# Autodesk Inventor assembly: tail_p1
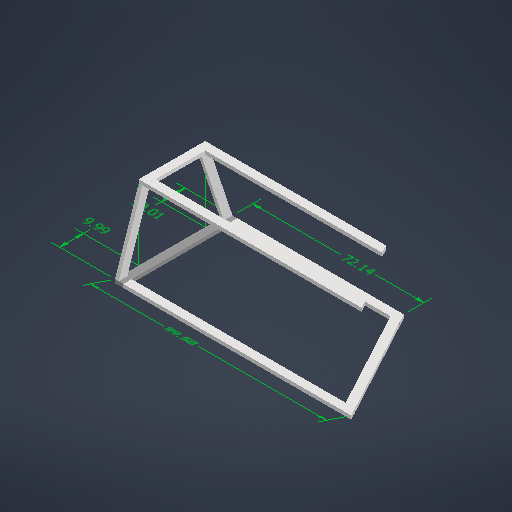
[picture p0: Inventor's stored thumbnail of the model, 512x512]
Saved by Autodesk Inventor 2027.1 (Build 311270010, 270A)
## iProperties
Created: 2026-09-01
Part Number: tail_p1
Document SubType Name: Assembly
Designer: jorda
Author: jorda
## Documents named in this file (9)
- C:\Users\jorda\OneDrive\Documents\GitHub\USC-ASME-TigerBurn-2026\CAD\Tail\tail_p1.iam
- C:\Users\jorda\OneDrive\Documents\GitHub\USC-ASME-TigerBurn-2026\CAD\Tail\2x4x48.ipt
- C:\Users\jorda\OneDrive\Documents\GitHub\USC-ASME-TigerBurn-2026\CAD\Tail\S_2x4x50.56.ipt
- C:\Users\jorda\OneDrive\Documents\GitHub\USC-ASME-TigerBurn-2026\CAD\Tail\S_2x4x72.ipt
- C:\Users\jorda\OneDrive\Documents\GitHub\USC-ASME-TigerBurn-2026\CAD\Tail\S_2x4x96.ipt
- C:\Users\jorda\OneDrive\Documents\GitHub\USC-ASME-TigerBurn-2026\CAD\Tail\S_2x4x32.93.ipt
- C:\Users\jorda\OneDrive\Documents\GitHub\USC-ASME-TigerBurn-2026\CAD\Tail\2x4x28.ipt
- C:\Users\jorda\OneDrive\Documents\GitHub\USC-ASME-TigerBurn-2026\CAD\Tail\S_2x4x93.85.ipt
- C:\Users\jorda\OneDrive\Documents\GitHub\USC-ASME-TigerBurn-2026\CAD\Tail\S_2x4x74.54.ipt
## Components (9 placed, 8 different names)
1. 2x4x48:1 — Mate:3, Flush:5, Flush:6, Mate:4, Flush:7, Flush:8, Mate:9, Flush:11, Mate:10, Flush:12
2. S_2x4x50.56:1
3. S_2x4x72:1 — Mate:3, Flush:5, Flush:6
4. S_2x4x96:1 — Mate:4, Flush:7, Flush:8
5. S_2x4x32.93:1 — Mate:9, Flush:11, Mate:11, Mate:12, Flush:13
6. S_2x4x32.93:2 — Mate:10, Flush:12
7. 2x4x28:1 — Mate:11, Mate:12, Flush:13, Mate:15, Flush:18, Flush:19, Mate:16, Flush:20, Flush:21, Mate:17, Flush:22, Flush:23
8. S_2x4x93.85:1 — Mate:15, Flush:18, Flush:19, Mate:16, Flush:20, Flush:21
9. S_2x4x74.54:1 — Mate:17, Flush:22, Flush:23
## Relationships (22: Flush 13, Mate 9)
- Mate:3: 2x4x48:1 ↔ S_2x4x72:1
- Flush:5: 2x4x48:1 ↔ S_2x4x72:1
- Flush:6: 2x4x48:1 ↔ S_2x4x72:1
- Mate:4: 2x4x48:1 ↔ S_2x4x96:1
- Flush:7: 2x4x48:1 ↔ S_2x4x96:1
- Flush:8: 2x4x48:1 ↔ S_2x4x96:1
- Mate:9: 2x4x48:1 ↔ S_2x4x32.93:1
- Flush:11: 2x4x48:1 ↔ S_2x4x32.93:1
- Mate:10: 2x4x48:1 ↔ S_2x4x32.93:2
- Flush:12: 2x4x48:1 ↔ S_2x4x32.93:2
- Mate:11: S_2x4x32.93:1 ↔ 2x4x28:1
- Mate:12: S_2x4x32.93:1 ↔ 2x4x28:1
- Flush:13: S_2x4x32.93:1 ↔ 2x4x28:1
- Mate:15: 2x4x28:1 ↔ S_2x4x93.85:1
- Flush:18: 2x4x28:1 ↔ S_2x4x93.85:1
- Flush:19: 2x4x28:1 ↔ S_2x4x93.85:1
- Mate:16: 2x4x28:1 ↔ S_2x4x93.85:1
- Flush:20: 2x4x28:1 ↔ S_2x4x93.85:1
- Flush:21: 2x4x28:1 ↔ S_2x4x93.85:1
- Mate:17: 2x4x28:1 ↔ S_2x4x74.54:1
- Flush:22: 2x4x28:1 ↔ S_2x4x74.54:1
- Flush:23: 2x4x28:1 ↔ S_2x4x74.54:1
